# Autodesk Inventor assembly: 00_X02598_LEGOmini_CityGuy
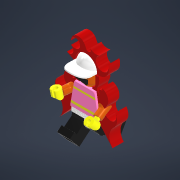
[picture p0: Inventor's stored thumbnail of the model, 180x180]
Saved by Autodesk Inventor 2022 (Build 260153000, 153)
## iProperties
Created: 2022-02-05
Part Number: 00_X02598_LEGOmini_CityGuy
Document SubType Name: Assembly
Designer: Jason
Author: Jason
## Documents named in this file (5)
- C:\Users\User\Desktop\110033226_LEGOmini_消防隊員\110033226_LEGOmini_消防隊員.iam
- C:\Users\User\Desktop\110033226_LEGOmini_消防隊員\110033226_LEGOmini_下半身.iam
- C:\Users\User\Desktop\110033226_LEGOmini_消防隊員\110033226_LEGOmini_上半身.iam
- C:\Users\User\Desktop\110033226_LEGOmini_消防隊員\110033226_LEGOmini_頭.ipt
- C:\Users\User\Desktop\110033226_LEGOmini_消防隊員\110033226_LEGOmini_帽子與火焰背景.ipt
## Components (4 placed, 4 different names)
1. 110033226_LEGOmini_下半身:1 [sub-assembly] — 貼合:1, 齊平:1, 齊平:2
2. 110033226_LEGOmini_上半身:1 [sub-assembly] — 貼合:1, 齊平:1, 齊平:2, 插入:1, 齊平:3
3. 110033226_LEGOmini_頭:1 — 插入:1, 插入:2, 齊平:3
4. 110033226_LEGOmini_帽子與火焰背景:1 — 插入:2
## Relationships (6: Flush 3, Insert 2, Mate 1)
- 貼合:1 [Mate]: 110033226_LEGOmini_下半身:1 ↔ 110033226_LEGOmini_上半身:1
- 齊平:1 [Flush]: 110033226_LEGOmini_下半身:1 ↔ 110033226_LEGOmini_上半身:1
- 齊平:2 [Flush]: 110033226_LEGOmini_下半身:1 ↔ 110033226_LEGOmini_上半身:1
- 插入:1 [Insert]: 110033226_LEGOmini_上半身:1 ↔ 110033226_LEGOmini_頭:1
- 插入:2 [Insert]: 110033226_LEGOmini_頭:1 ↔ 110033226_LEGOmini_帽子與火焰背景:1
- 齊平:3 [Flush]: 110033226_LEGOmini_上半身:1 ↔ 110033226_LEGOmini_頭:1
